# Autodesk Inventor assembly: Table
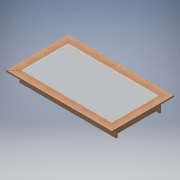
[picture p0: Inventor's stored thumbnail of the model, 180x180]
Saved by Autodesk Inventor 2016 (Build 200138000, 138)
## iProperties
Created: 2016-02-08
Part Number: Table
Document SubType Name: Assembly
Designer: ron
Mass: 50986 g
Surface Area: 141310 cm^2
Volume: 60602.2 cm^3
Density: 0.841322 g/cm^3
Author: ron
## Documents named in this file (14)
- E:\CAD\Table.iam
- E:\CAD\Parts\LedBoard.ipt
- E:\CAD\Parts\Acrylitep95.ipt
- E:\CAD\Parts\Glass.ipt
- E:\CAD\Parts\Bottom.ipt
- E:\CAD\Parts\PowerSupply.ipt
- E:\CAD\Parts\DividerWidthPlastic.ipt
- E:\CAD\Parts\DividerLengthPlastic.ipt
- E:\CAD\Parts\SkirtLength.ipt
- E:\CAD\Parts\SkirtWidth.ipt
- E:\CAD\Parts\SupportWedge.ipt
- E:\CAD\Parts\SkinnySideW.ipt
- E:\CAD\Parts\SkinnySideL.ipt
- E:\CAD\Parts\SkinnySideWOpposite.ipt
## Components (61 placed, 13 different names)
1. LedBoard:1 — Flush:127, Flush:128, Mate:93, Mate:94, Flush:138, Flush:139, Flush:140, Flush:141, Flush:143, Flush:144, Flush:146, Flush:147, Flush:149, Flush:150, Flush:152, Flush:153, Flush:155, Flush:156, Flush:158, Flush:159, Flush:161, Flush:162, Flush:164, Flush:165, Flush:167, Flush:168, Flush:170, Flush:171, Flush:173, Flush:174, Flush:176, Flush:177, Flush:179, Flush:180, Flush:182, Flush:183, Flush:185, Flush:186, Flush:188, Flush:189, Flush:191, Flush:192, Flush:194, Flush:195, Flush:197, Flush:198, Flush:200, Flush:201, Flush:203, Flush:204, Flush:206, Flush:207, Flush:209, Flush:210, Flush:212, Flush:213, Flush:215, Flush:216, Flush:218, Flush:220, Flush:221, Flush:223, Flush:224, Flush:226, Flush:227, Flush:229, Mate:95, Flush:230, Flush:231, Mate:96, Flush:232, Mate:97, Flush:234, Mate:98, Flush:236, Mate:99, Flush:238, Mate:100, Flush:240, Mate:101, Flush:242, Mate:102, Flush:244, Mate:103, Flush:246, Mate:104, Flush:249, Mate:105, Flush:251, Mate:106, Flush:253, Mate:107, Flush:255, Mate:108, Flush:257, Mate:109, Flush:259, Mate:171, Flush:260, Mate:173, Mate:177, Mate:178, Mate:180, Mate:183, Mate:185
2. Acrylitep95:1 — Flush:127, Flush:128, Mate:20, Flush:129, Flush:130, Mate:93, Mate:117, Mate:119, Mate:122, Mate:125
3. Glass:1 — Mate:20, Flush:129, Flush:130, Mate:118, Mate:121, Mate:124
4. Bottom:1 — Flush:131, Flush:132, Mate:170, Flush:262, Mate:182, Flush:263, Mate:186, Flush:264, Flush:265, Mate:187, Flush:266, Flush:267
5. PowerSupply:1 — Flush:131, Flush:132, Mate:170
6. DividerWidthPlastic:1 — Flush:161, Flush:162, Flush:163, Flush:166
7. DividerWidthPlastic:2 — Flush:167, Flush:168, Flush:169, Flush:172
8. DividerWidthPlastic:3 — Flush:176, Flush:177, Flush:178, Flush:181
9. DividerWidthPlastic:4 — Flush:215, Flush:216, Flush:217, Flush:219
10. DividerWidthPlastic:6 — Flush:170, Flush:171, Flush:172, Flush:175
11. DividerWidthPlastic:7 — Flush:164, Flush:165, Flush:166, Flush:169
12. DividerWidthPlastic:8 — Flush:155, Flush:156, Flush:157, Flush:160
13. DividerWidthPlastic:9 — Flush:158, Flush:159, Flush:160, Flush:163
14. DividerWidthPlastic:10 — Flush:188, Flush:189, Flush:190, Flush:193
15. DividerWidthPlastic:11 — Flush:212, Flush:213, Flush:214, Flush:217
16. DividerWidthPlastic:12 — Flush:218, Flush:219, Flush:220, Flush:222
17. DividerWidthPlastic:13 — Flush:185, Flush:186, Flush:187, Flush:190
18. DividerWidthPlastic:14 — Flush:182, Flush:183, Flush:184, Flush:187
19. DividerWidthPlastic:15 — Flush:179, Flush:180, Flush:181, Flush:184
20. DividerWidthPlastic:16 — Flush:200, Flush:201, Flush:202, Flush:205
21. DividerWidthPlastic:17 — Flush:194, Flush:195, Flush:196, Flush:199
22. DividerWidthPlastic:18 — Flush:191, Flush:192, Flush:193, Flush:196
23. DividerWidthPlastic:19 — Flush:197, Flush:198, Flush:199, Flush:202
24. DividerWidthPlastic:20 — Flush:209, Flush:210, Flush:211, Flush:214
25. DividerWidthPlastic:21 — Mate:94, Flush:138, Flush:139, Flush:142
26. DividerWidthPlastic:22 — Flush:149, Flush:150, Flush:151, Flush:154
27. DividerWidthPlastic:23 — Flush:206, Flush:207, Flush:208, Flush:211
28. DividerWidthPlastic:24 — Flush:140, Flush:141, Flush:142, Flush:145, Mate:120
29. DividerWidthPlastic:25 — Flush:203, Flush:204, Flush:205, Flush:208
30. DividerWidthPlastic:26 — Flush:143, Flush:144, Flush:145, Flush:148
31. DividerWidthPlastic:27 — Flush:146, Flush:147, Flush:148, Flush:151
32. DividerWidthPlastic:28 — Flush:152, Flush:153, Flush:154, Flush:157
33. DividerWidthPlastic:29 — Flush:221, Flush:222, Flush:223, Flush:225
34. DividerWidthPlastic:30 — Flush:224, Flush:225, Flush:226, Flush:228
35. DividerWidthPlastic:31 — Flush:227, Flush:228, Flush:229
36. DividerWidthPlastic:32 — Flush:173, Flush:174, Flush:175, Flush:178
37. DividerLengthPlastic:1 — Mate:95, Flush:230, Flush:231, Flush:233
38. DividerLengthPlastic:2 — Mate:98, Flush:236, Flush:237, Flush:239
39. DividerLengthPlastic:3 — Mate:99, Flush:238, Flush:239, Flush:241
40. DividerLengthPlastic:4 — Mate:104, Flush:248, Flush:249, Flush:250
41. DividerLengthPlastic:5 — Mate:107, Flush:254, Flush:255, Flush:256
42. DividerLengthPlastic:7 — Mate:109, Flush:258, Flush:259
43. DividerLengthPlastic:8 — Mate:105, Flush:250, Flush:251, Flush:252
44. DividerLengthPlastic:9 — Mate:103, Flush:246, Flush:247, Flush:248
45. DividerLengthPlastic:10 — Mate:101, Flush:242, Flush:243, Flush:245
46. DividerLengthPlastic:11 — Mate:97, Flush:234, Flush:235, Flush:237
47. DividerLengthPlastic:12 — Mate:96, Flush:232, Flush:233, Flush:235
48. DividerLengthPlastic:13 — Mate:100, Flush:240, Flush:241, Flush:243
49. DividerLengthPlastic:14 — Mate:102, Flush:244, Flush:245, Flush:247
50. DividerLengthPlastic:15 — Mate:106, Flush:252, Flush:253, Flush:254, Mate:123
51. DividerLengthPlastic:17 — Mate:108, Flush:256, Flush:257, Flush:258, Mate:116
52. SkirtLength:1 — Mate:119, Mate:120, Mate:121
53. SkirtLength:2 — Mate:125, Mate:126, Mate:127
54. SkirtWidth:1 — Mate:116, Mate:117, Mate:118, Mate:127
55. SkirtWidth:2 — Mate:122, Mate:123, Mate:124, Mate:126
56. SupportWedge:1 — Mate:186, Flush:264, Flush:265
57. SupportWedge:2 — Mate:187, Flush:266, Flush:267
58. SkinnySideW:1 — Mate:173, Mate:177, Mate:179, Flush:261, Mate:181, Flush:262, Flush:263
59. SkinnySideL:1 — Mate:171, Flush:260, Mate:178, Mate:179, Mate:182
60. SkinnySideL:2 — Mate:180, Flush:261, Mate:181, Mate:184
61. SkinnySideWOpposite:1 — Mate:183, Mate:184, Mate:185
## Relationships (180: Flush 136, Mate 44)
- Flush:127 (-25.4 mm): LedBoard:1 ↔ Acrylitep95:1
- Flush:128 (-25.4 mm): LedBoard:1 ↔ Acrylitep95:1
- Mate:20: Acrylitep95:1 ↔ Glass:1
- Flush:129: Acrylitep95:1 ↔ Glass:1
- Flush:130: Acrylitep95:1 ↔ Glass:1
- Flush:131 (50.8 mm): Bottom:1 ↔ PowerSupply:1
- Flush:132 (50.8 mm): Bottom:1 ↔ PowerSupply:1
- Mate:93 (50.8 mm): LedBoard:1 ↔ Acrylitep95:1
- Mate:94: LedBoard:1 ↔ DividerWidthPlastic:21
- Flush:138: LedBoard:1 ↔ DividerWidthPlastic:21
- Flush:139 (36.5125 mm): LedBoard:1 ↔ DividerWidthPlastic:21
- Flush:140 (-50.8 mm): LedBoard:1 ↔ DividerWidthPlastic:24
- Flush:141: LedBoard:1 ↔ DividerWidthPlastic:24
- Flush:142 (38.1 mm): DividerWidthPlastic:21 ↔ DividerWidthPlastic:24
- Flush:143 (-50.8 mm): LedBoard:1 ↔ DividerWidthPlastic:26
- Flush:144: LedBoard:1 ↔ DividerWidthPlastic:26
- Flush:145 (38.1 mm): DividerWidthPlastic:24 ↔ DividerWidthPlastic:26
- Flush:146 (-50.8 mm): LedBoard:1 ↔ DividerWidthPlastic:27
- Flush:147: LedBoard:1 ↔ DividerWidthPlastic:27
- Flush:148 (38.1 mm): DividerWidthPlastic:26 ↔ DividerWidthPlastic:27
- Flush:149 (-50.8 mm): LedBoard:1 ↔ DividerWidthPlastic:22
- Flush:150: LedBoard:1 ↔ DividerWidthPlastic:22
- Flush:151 (38.1 mm): DividerWidthPlastic:22 ↔ DividerWidthPlastic:27
- Flush:152 (-50.8 mm): LedBoard:1 ↔ DividerWidthPlastic:28
- Flush:153: LedBoard:1 ↔ DividerWidthPlastic:28
- Flush:154 (38.1 mm): DividerWidthPlastic:22 ↔ DividerWidthPlastic:28
- Flush:155 (-50.8 mm): LedBoard:1 ↔ DividerWidthPlastic:8
- Flush:156: LedBoard:1 ↔ DividerWidthPlastic:8
- Flush:157 (38.1 mm): DividerWidthPlastic:8 ↔ DividerWidthPlastic:28
- Flush:158 (-50.8 mm): LedBoard:1 ↔ DividerWidthPlastic:9
- Flush:159: LedBoard:1 ↔ DividerWidthPlastic:9
- Flush:160 (38.1 mm): DividerWidthPlastic:8 ↔ DividerWidthPlastic:9
- Flush:161 (-50.8 mm): LedBoard:1 ↔ DividerWidthPlastic:1
- Flush:162: LedBoard:1 ↔ DividerWidthPlastic:1
- Flush:163 (38.1 mm): DividerWidthPlastic:1 ↔ DividerWidthPlastic:9
- Flush:164 (-50.8 mm): LedBoard:1 ↔ DividerWidthPlastic:7
- Flush:165: LedBoard:1 ↔ DividerWidthPlastic:7
- Flush:166 (38.1 mm): DividerWidthPlastic:1 ↔ DividerWidthPlastic:7
- Flush:167 (-50.8 mm): LedBoard:1 ↔ DividerWidthPlastic:2
- Flush:168: LedBoard:1 ↔ DividerWidthPlastic:2
- Flush:169 (38.1 mm): DividerWidthPlastic:2 ↔ DividerWidthPlastic:7
- Flush:170 (-50.8 mm): LedBoard:1 ↔ DividerWidthPlastic:6
- Flush:171: LedBoard:1 ↔ DividerWidthPlastic:6
- Flush:172 (38.1 mm): DividerWidthPlastic:2 ↔ DividerWidthPlastic:6
- Flush:173 (-50.8 mm): LedBoard:1 ↔ DividerWidthPlastic:32
- Flush:174: LedBoard:1 ↔ DividerWidthPlastic:32
- Flush:175 (38.1 mm): DividerWidthPlastic:6 ↔ DividerWidthPlastic:32
- Flush:176 (-50.8 mm): LedBoard:1 ↔ DividerWidthPlastic:3
- Flush:177: LedBoard:1 ↔ DividerWidthPlastic:3
- Flush:178 (38.1 mm): DividerWidthPlastic:3 ↔ DividerWidthPlastic:32
- Flush:179 (-50.8 mm): LedBoard:1 ↔ DividerWidthPlastic:15
- Flush:180: LedBoard:1 ↔ DividerWidthPlastic:15
- Flush:181 (38.1 mm): DividerWidthPlastic:3 ↔ DividerWidthPlastic:15
- Flush:182 (-50.8 mm): LedBoard:1 ↔ DividerWidthPlastic:14
- Flush:183: LedBoard:1 ↔ DividerWidthPlastic:14
- Flush:184 (38.1 mm): DividerWidthPlastic:14 ↔ DividerWidthPlastic:15
- Flush:185 (-50.8 mm): LedBoard:1 ↔ DividerWidthPlastic:13
- Flush:186: LedBoard:1 ↔ DividerWidthPlastic:13
- Flush:187 (38.1 mm): DividerWidthPlastic:13 ↔ DividerWidthPlastic:14
- Flush:188 (-50.8 mm): LedBoard:1 ↔ DividerWidthPlastic:10
- Flush:189: LedBoard:1 ↔ DividerWidthPlastic:10
- Flush:190 (38.1 mm): DividerWidthPlastic:10 ↔ DividerWidthPlastic:13
- Flush:191 (-50.8 mm): LedBoard:1 ↔ DividerWidthPlastic:18
- Flush:192: LedBoard:1 ↔ DividerWidthPlastic:18
- Flush:193 (38.1 mm): DividerWidthPlastic:10 ↔ DividerWidthPlastic:18
- Flush:194 (-50.8 mm): LedBoard:1 ↔ DividerWidthPlastic:17
- Flush:195: LedBoard:1 ↔ DividerWidthPlastic:17
- Flush:196 (38.1 mm): DividerWidthPlastic:17 ↔ DividerWidthPlastic:18
- Flush:197 (-50.8 mm): LedBoard:1 ↔ DividerWidthPlastic:19
- Flush:198: LedBoard:1 ↔ DividerWidthPlastic:19
- Flush:199 (38.1 mm): DividerWidthPlastic:17 ↔ DividerWidthPlastic:19
- Flush:200 (-50.8 mm): LedBoard:1 ↔ DividerWidthPlastic:16
- Flush:201: LedBoard:1 ↔ DividerWidthPlastic:16
- Flush:202 (38.1 mm): DividerWidthPlastic:16 ↔ DividerWidthPlastic:19
- Flush:203 (-50.8 mm): LedBoard:1 ↔ DividerWidthPlastic:25
- Flush:204: LedBoard:1 ↔ DividerWidthPlastic:25
- Flush:205 (38.1 mm): DividerWidthPlastic:16 ↔ DividerWidthPlastic:25
- Flush:206 (-50.8 mm): LedBoard:1 ↔ DividerWidthPlastic:23
- Flush:207: LedBoard:1 ↔ DividerWidthPlastic:23
- Flush:208 (38.1 mm): DividerWidthPlastic:23 ↔ DividerWidthPlastic:25
- Flush:209 (-50.8 mm): LedBoard:1 ↔ DividerWidthPlastic:20
- Flush:210: LedBoard:1 ↔ DividerWidthPlastic:20
- Flush:211 (38.1 mm): DividerWidthPlastic:20 ↔ DividerWidthPlastic:23
- Flush:212 (-50.8 mm): LedBoard:1 ↔ DividerWidthPlastic:11
- Flush:213: LedBoard:1 ↔ DividerWidthPlastic:11
- Flush:214 (38.1 mm): DividerWidthPlastic:11 ↔ DividerWidthPlastic:20
- Flush:215 (-50.8 mm): LedBoard:1 ↔ DividerWidthPlastic:4
- Flush:216: LedBoard:1 ↔ DividerWidthPlastic:4
- Flush:217 (38.1 mm): DividerWidthPlastic:4 ↔ DividerWidthPlastic:11
- Flush:218 (-50.8 mm): LedBoard:1 ↔ DividerWidthPlastic:12
- Flush:219 (38.1 mm): DividerWidthPlastic:4 ↔ DividerWidthPlastic:12
- Flush:220: LedBoard:1 ↔ DividerWidthPlastic:12
- Flush:221 (-50.8 mm): LedBoard:1 ↔ DividerWidthPlastic:29
- Flush:222 (38.1 mm): DividerWidthPlastic:12 ↔ DividerWidthPlastic:29
- Flush:223: LedBoard:1 ↔ DividerWidthPlastic:29
- Flush:224 (-50.8 mm): LedBoard:1 ↔ DividerWidthPlastic:30
- Flush:225 (38.1 mm): DividerWidthPlastic:29 ↔ DividerWidthPlastic:30
- Flush:226: LedBoard:1 ↔ DividerWidthPlastic:30
- Flush:227 (-50.8 mm): LedBoard:1 ↔ DividerWidthPlastic:31
- Flush:228 (38.1 mm): DividerWidthPlastic:30 ↔ DividerWidthPlastic:31
- Flush:229: LedBoard:1 ↔ DividerWidthPlastic:31
- Mate:95: LedBoard:1 ↔ DividerLengthPlastic:1
- Flush:230: LedBoard:1 ↔ DividerLengthPlastic:1
- Flush:231 (36.5125 mm): LedBoard:1 ↔ DividerLengthPlastic:1
- Mate:96: LedBoard:1 ↔ DividerLengthPlastic:12
- Flush:232: LedBoard:1 ↔ DividerLengthPlastic:12
- Flush:233 (-38.1 mm): DividerLengthPlastic:1 ↔ DividerLengthPlastic:12
- Mate:97: LedBoard:1 ↔ DividerLengthPlastic:11
- Flush:234: LedBoard:1 ↔ DividerLengthPlastic:11
- Flush:235 (38.1 mm): DividerLengthPlastic:11 ↔ DividerLengthPlastic:12
- Mate:98: LedBoard:1 ↔ DividerLengthPlastic:2
- Flush:236: LedBoard:1 ↔ DividerLengthPlastic:2
- Flush:237 (38.1 mm): DividerLengthPlastic:2 ↔ DividerLengthPlastic:11
- Mate:99: LedBoard:1 ↔ DividerLengthPlastic:3
- Flush:238: LedBoard:1 ↔ DividerLengthPlastic:3
- Flush:239 (38.1 mm): DividerLengthPlastic:2 ↔ DividerLengthPlastic:3
- Mate:100: LedBoard:1 ↔ DividerLengthPlastic:13
- Flush:240: LedBoard:1 ↔ DividerLengthPlastic:13
- Flush:241 (38.1 mm): DividerLengthPlastic:3 ↔ DividerLengthPlastic:13
- Mate:101: LedBoard:1 ↔ DividerLengthPlastic:10
- Flush:242: LedBoard:1 ↔ DividerLengthPlastic:10
- Flush:243 (38.1 mm): DividerLengthPlastic:10 ↔ DividerLengthPlastic:13
- Mate:102: LedBoard:1 ↔ DividerLengthPlastic:14
- Flush:244: LedBoard:1 ↔ DividerLengthPlastic:14
- Flush:245 (38.1 mm): DividerLengthPlastic:10 ↔ DividerLengthPlastic:14
- Mate:103: LedBoard:1 ↔ DividerLengthPlastic:9
- Flush:246: LedBoard:1 ↔ DividerLengthPlastic:9
- Flush:247 (38.1 mm): DividerLengthPlastic:9 ↔ DividerLengthPlastic:14
- Mate:104: LedBoard:1 ↔ DividerLengthPlastic:4
- Flush:248 (38.1 mm): DividerLengthPlastic:4 ↔ DividerLengthPlastic:9
- Flush:249: LedBoard:1 ↔ DividerLengthPlastic:4
- Mate:105: LedBoard:1 ↔ DividerLengthPlastic:8
- Flush:250 (38.1 mm): DividerLengthPlastic:4 ↔ DividerLengthPlastic:8
- Flush:251: LedBoard:1 ↔ DividerLengthPlastic:8
- Mate:106: LedBoard:1 ↔ DividerLengthPlastic:15
- Flush:252 (38.1 mm): DividerLengthPlastic:8 ↔ DividerLengthPlastic:15
- Flush:253: LedBoard:1 ↔ DividerLengthPlastic:15
- Mate:107: LedBoard:1 ↔ DividerLengthPlastic:5
- Flush:254 (38.1 mm): DividerLengthPlastic:5 ↔ DividerLengthPlastic:15
- Flush:255: LedBoard:1 ↔ DividerLengthPlastic:5
- Mate:108: LedBoard:1 ↔ DividerLengthPlastic:17
- Flush:256 (38.1 mm): DividerLengthPlastic:5 ↔ DividerLengthPlastic:17
- Flush:257: LedBoard:1 ↔ DividerLengthPlastic:17
- Mate:109: LedBoard:1 ↔ DividerLengthPlastic:7
- Flush:258 (38.1 mm): DividerLengthPlastic:7 ↔ DividerLengthPlastic:17
- Flush:259: LedBoard:1 ↔ DividerLengthPlastic:7
- Mate:116: DividerLengthPlastic:17 ↔ SkirtWidth:1
- Mate:117: Acrylitep95:1 ↔ SkirtWidth:1
- Mate:118: Glass:1 ↔ SkirtWidth:1
- Mate:119: Acrylitep95:1 ↔ SkirtLength:1
- Mate:120: DividerWidthPlastic:24 ↔ SkirtLength:1
- Mate:121: Glass:1 ↔ SkirtLength:1
- Mate:122: Acrylitep95:1 ↔ SkirtWidth:2
- Mate:123: DividerLengthPlastic:15 ↔ SkirtWidth:2
- Mate:124: Glass:1 ↔ SkirtWidth:2
- Mate:125: Acrylitep95:1 ↔ SkirtLength:2
- Mate:126: SkirtLength:2 ↔ SkirtWidth:2
- Mate:127: SkirtLength:2 ↔ SkirtWidth:1
- Mate:170: Bottom:1 ↔ PowerSupply:1
- Mate:171: LedBoard:1 ↔ SkinnySideL:1
- Flush:260 (-60.7924 mm): LedBoard:1 ↔ SkinnySideL:1
- Mate:173: LedBoard:1 ↔ SkinnySideW:1
- Mate:177: LedBoard:1 ↔ SkinnySideW:1
- Mate:178: LedBoard:1 ↔ SkinnySideL:1
- Mate:179: SkinnySideW:1 ↔ SkinnySideL:1
- Mate:180: LedBoard:1 ↔ SkinnySideL:2
- Flush:261 (-50.8 mm): SkinnySideW:1 ↔ SkinnySideL:2
- Mate:181: SkinnySideW:1 ↔ SkinnySideL:2
- Flush:262: Bottom:1 ↔ SkinnySideW:1
- Mate:182: Bottom:1 ↔ SkinnySideL:1
- Flush:263 (6.35 mm): Bottom:1 ↔ SkinnySideW:1
- Mate:183: LedBoard:1 ↔ SkinnySideWOpposite:1
- Mate:184: SkinnySideL:2 ↔ SkinnySideWOpposite:1
- Mate:185: LedBoard:1 ↔ SkinnySideWOpposite:1
- Mate:186: Bottom:1 ↔ SupportWedge:1
- Flush:264: Bottom:1 ↔ SupportWedge:1
- Flush:265: Bottom:1 ↔ SupportWedge:1
- Mate:187: Bottom:1 ↔ SupportWedge:2
- Flush:266: Bottom:1 ↔ SupportWedge:2
- Flush:267: Bottom:1 ↔ SupportWedge:2
